# Autodesk Inventor assembly: Chain Drive
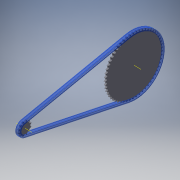
[picture p0: Inventor's stored thumbnail of the model, 180x180]
Saved by Autodesk Inventor 2016 (Build 200138000, 138)
## iProperties
ClientObjectVersion: 1
Created: 2016-05-21
Part Number: Chain Drive
Document SubType Name: Assembly
Designer: Henrik Samuelsson
Author: Henrik Samuelsson
## Documents named in this file (4)
- C:\Users\Henrik Samuelsson\Documents\Killer-Bot-2016\AutodeskWorkspace\57mmTest\Design Accelerator\Chain Drive3.iam
- C:\Users\Henrik Samuelsson\Documents\Killer-Bot-2016\AutodeskWorkspace\57mmTest\Design Accelerator\Roller Chain3.ipt
- C:\Users\Henrik Samuelsson\Documents\Killer-Bot-2016\AutodeskWorkspace\57mmTest\Design Accelerator\Roller Chain Sprocket13.ipt
- C:\Users\Henrik Samuelsson\Documents\Killer-Bot-2016\AutodeskWorkspace\57mmTest\Design Accelerator\Roller Chain Sprocket23.ipt
## Components (3 placed, 3 different names)
1. Roller Chain:1 — Flush:1, Mate:1, Mate:2, Flush:2, Mate:3, Mate:4
2. Roller Chain Sprocket1:1 — Flush:1, Mate:1, Mate:2, Rotation:1
3. Roller Chain Sprocket2:1 — Flush:2, Mate:3, Rotation:1, Mate:4
## Relationships (7: Mate 4, Flush 2, RelateRotation 1)
- Flush:1: Roller Chain:1 ↔ Roller Chain Sprocket1:1
- Mate:1: Roller Chain:1 ↔ Roller Chain Sprocket1:1
- Mate:2: Roller Chain:1 ↔ Roller Chain Sprocket1:1
- Flush:2: Roller Chain:1 ↔ Roller Chain Sprocket2:1
- Mate:3: Roller Chain:1 ↔ Roller Chain Sprocket2:1
- Rotation:1 [RelateRotation] (4.75 ul): Roller Chain Sprocket1:1 ↔ Roller Chain Sprocket2:1
- Mate:4: Roller Chain:1 ↔ Roller Chain Sprocket2:1
